# Autodesk Inventor assembly: Field_Assy
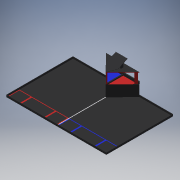
[picture p0: Inventor's stored thumbnail of the model, 180x180]
Saved by Autodesk Inventor 2017 (Build 210142000, 142)
## iProperties
Created: 2017-04-14
Part Number: Field_Assy
Document SubType Name: Assembly
Designer: Alex Tacescu
Author: Alex Tacescu
## Documents named in this file (3)
- C:\Users\alext\Documents\School\WPI\Spring 2017\RBE 1001\Final Project\Field Parts\Field_Assy.iam
- C:\Users\alext\Documents\School\WPI\Spring 2017\RBE 1001\Final Project\Field Parts\Field.ipt
- C:\Users\alext\Documents\School\WPI\Spring 2017\RBE 1001\Final Project\Field Parts\Barn and Rad.ipt
## Components (2 placed, 2 different names)
1. Field:1 — Flush:1, Flush:2, Flush:3, Mate:1, Mate:2
2. Barn and Rad:1 — Mate:1, Mate:2, Flush:4
## Relationships (6: Flush 4, Mate 2)
- Flush:1: Field:1
- Flush:2: Field:1
- Flush:3: Field:1
- Mate:1: Field:1 ↔ Barn and Rad:1
- Mate:2: Field:1 ↔ Barn and Rad:1
- Flush:4: Barn and Rad:1
